# Autodesk Inventor assembly: Calorímetro
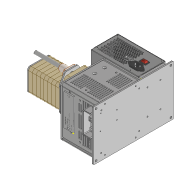
[picture p0: Inventor's stored thumbnail of the model, 180x180]
Saved by Autodesk Inventor 2020 (Build 240168000, 168)
## iProperties
Created: 2022-07-16
Part Number: Calorímetro
Document SubType Name: Assembly
Designer: gabri
Author: gabri
## Documents named in this file (15)
- C:\Users\gabri\OneDrive\Área de Trabalho\Calorimetro 2022\Calorimetro github\Inventor\Calorímetro.iam
- C:\Users\gabri\OneDrive\Área de Trabalho\Calorimetro 2022\Calorimetro github\Inventor\Fonte\ATX Power Supply v1.iam
- C:\Users\gabri\OneDrive\Área de Trabalho\Calorimetro 2022\Calorimetro github\Inventor\Base.ipt
- C:\Users\gabri\OneDrive\Área de Trabalho\Calorimetro 2022\Calorimetro github\Inventor\parte_superior.iam
- C:\Users\gabri\OneDrive\Área de Trabalho\Calorimetro 2022\Calorimetro github\Inventor\Montagem_suporte_termopar.iam
- C:\Users\gabri\OneDrive\Área de Trabalho\Calorimetro 2022\Calorimetro github\Inventor\Peça4.ipt
- C:\Users\gabri\OneDrive\Área de Trabalho\Calorimetro 2022\Calorimetro github\Inventor\suporte-fonte.ipt
- C:\Users\gabri\OneDrive\Área de Trabalho\Calorimetro 2022\Calorimetro github\Inventor\suporte_fechamento.ipt
- C:\Users\gabri\OneDrive\Área de Trabalho\Calorimetro 2022\Calorimetro github\Inventor\fechamentocima.ipt
- C:\Users\gabri\OneDrive\Área de Trabalho\Calorimetro 2022\Calorimetro github\Inventor\Mega.ipt
- C:\Users\gabri\OneDrive\Área de Trabalho\Calorimetro 2022\Calorimetro github\Inventor\suporte_fechamento_tipo2.ipt
- C:\Users\gabri\OneDrive\Área de Trabalho\Calorimetro 2022\Calorimetro github\Inventor\fechamento1.ipt
- C:\Users\gabri\OneDrive\Área de Trabalho\Calorimetro 2022\Calorimetro github\Inventor\fechamento2.ipt
- C:\Users\gabri\OneDrive\Área de Trabalho\Calorimetro 2022\Calorimetro github\Inventor\Placa.ipt
- C:\Users\gabri\OneDrive\Área de Trabalho\Calorimetro 2022\Calorimetro github\Inventor\Montagem_corpo_menor.iam
## Components (17 placed, 14 different names)
1. ATX Power Supply v1:1 [sub-assembly] — Coincidência:1, Alinhamento:1, Coincidência:2, Coincidência:5, Coincidência:6, Alinhamento:4, Alinhamento:5, Alinhamento:6, Alinhamento:7
2. Base:1 — Coincidência:7, Alinhamento:6, Alinhamento:7, Coincidência:8, Coincidência:9, Alinhamento:8, Alinhamento:9, Alinhamento:10, Coincidência:16, Alinhamento:19, Alinhamento:20, Coincidência:24
3. parte_superior:1 [sub-assembly] — Coincidência:4, Alinhamento:2, Coincidência:13, Alinhamento:17, Alinhamento:18, Coincidência:14, Coincidência:29, Coincidência:30
4. Montagem_suporte_termopar:1 [sub-assembly] — Coincidência:4, Coincidência:14, Coincidência:15, Ângulo:1
5. Peça4:1 — Alinhamento:2
6. suporte-fonte:1 — Coincidência:5, Coincidência:6, Coincidência:7, Alinhamento:4, Alinhamento:5
7. suporte_fechamento:1 — Coincidência:8, Alinhamento:8, Alinhamento:11, Alinhamento:15, Coincidência:23, Coincidência:28
8. suporte_fechamento:2 — Coincidência:9, Alinhamento:9, Alinhamento:10, Alinhamento:11, Alinhamento:16, Alinhamento:21, Alinhamento:22
9. fechamentocima:1 — Alinhamento:15, Alinhamento:16, Coincidência:13, Alinhamento:17, Alinhamento:18, Coincidência:15, Ângulo:1, Coincidência:17, Coincidência:18, Coincidência:19, Coincidência:20, Coincidência:21, Coincidência:22, Coincidência:27
10. Mega:1 — Coincidência:16, Alinhamento:19, Alinhamento:20
11. suporte_fechamento_tipo2:1 — Coincidência:17, Coincidência:18, Coincidência:19, Coincidência:26
12. suporte_fechamento:3 — Coincidência:20, Coincidência:21, Coincidência:22
13. fechamento1:1 — Alinhamento:21, Alinhamento:22
14. fechamento2:1 — Coincidência:23, Coincidência:24, Coincidência:25
15. Placa:1 — Coincidência:25
16. fechamento1:2 — Coincidência:26, Coincidência:27, Coincidência:28
17. Montagem_corpo_menor:1 [sub-assembly] — Coincidência:29, Coincidência:30
## Relationships (45: Mate 26, Flush 18, Angle 1)
- Coincidência:1 [Mate] (-71 mm): ATX Power Supply v1:1
- Alinhamento:1 [Flush]: ATX Power Supply v1:1
- Coincidência:2 [Mate]: ATX Power Supply v1:1
- Coincidência:4 [Mate]: parte_superior:1 ↔ Montagem_suporte_termopar:1
- Alinhamento:2 [Flush]: parte_superior:1 ↔ Peça4:1
- Coincidência:5 [Mate]: ATX Power Supply v1:1 ↔ suporte-fonte:1
- Coincidência:6 [Mate]: ATX Power Supply v1:1 ↔ suporte-fonte:1
- Coincidência:7 [Mate]: Base:1 ↔ suporte-fonte:1
- Alinhamento:4 [Flush]: ATX Power Supply v1:1 ↔ suporte-fonte:1
- Alinhamento:5 [Flush] (-8 mm): ATX Power Supply v1:1 ↔ suporte-fonte:1
- Alinhamento:6 [Flush] (-13 mm): ATX Power Supply v1:1 ↔ Base:1
- Alinhamento:7 [Flush]: ATX Power Supply v1:1 ↔ Base:1
- Coincidência:8 [Mate]: Base:1 ↔ suporte_fechamento:1
- Coincidência:9 [Mate]: Base:1 ↔ suporte_fechamento:2
- Alinhamento:8 [Flush]: Base:1 ↔ suporte_fechamento:1
- Alinhamento:9 [Flush]: Base:1 ↔ suporte_fechamento:2
- Alinhamento:10 [Flush] (15 mm): Base:1 ↔ suporte_fechamento:2
- Alinhamento:11 [Flush]: suporte_fechamento:1 ↔ suporte_fechamento:2
- Alinhamento:15 [Flush]: suporte_fechamento:1 ↔ fechamentocima:1
- Alinhamento:16 [Flush]: suporte_fechamento:2 ↔ fechamentocima:1
- Coincidência:13 [Mate]: parte_superior:1 ↔ fechamentocima:1
- Alinhamento:17 [Flush] (33.5 mm): parte_superior:1 ↔ fechamentocima:1
- Alinhamento:18 [Flush] (12.82 mm): parte_superior:1 ↔ fechamentocima:1
- Coincidência:14 [Mate]: parte_superior:1 ↔ Montagem_suporte_termopar:1
- Coincidência:15 [Mate]: Montagem_suporte_termopar:1 ↔ fechamentocima:1
- Ângulo:1 [Angle] (0 deg): Montagem_suporte_termopar:1 ↔ fechamentocima:1
- Coincidência:16 [Mate]: Base:1 ↔ Mega:1
- Alinhamento:19 [Flush] (3 mm): Base:1 ↔ Mega:1
- Alinhamento:20 [Flush] (26 mm): Base:1 ↔ Mega:1
- Coincidência:17 [Mate]: fechamentocima:1 ↔ suporte_fechamento_tipo2:1
- Coincidência:18 [Mate]: fechamentocima:1 ↔ suporte_fechamento_tipo2:1
- Coincidência:19 [Mate]: fechamentocima:1 ↔ suporte_fechamento_tipo2:1
- Coincidência:20 [Mate]: fechamentocima:1 ↔ suporte_fechamento:3
- Coincidência:21 [Mate]: fechamentocima:1 ↔ suporte_fechamento:3
- Coincidência:22 [Mate]: fechamentocima:1 ↔ suporte_fechamento:3
- Alinhamento:21 [Flush]: suporte_fechamento:2 ↔ fechamento1:1
- Alinhamento:22 [Flush]: suporte_fechamento:2 ↔ fechamento1:1
- Coincidência:23 [Mate]: suporte_fechamento:1 ↔ fechamento2:1
- Coincidência:24 [Mate]: Base:1 ↔ fechamento2:1
- Coincidência:25 [Mate]: fechamento2:1 ↔ Placa:1
- Coincidência:26 [Mate]: suporte_fechamento_tipo2:1 ↔ fechamento1:2
- Coincidência:27 [Mate]: fechamentocima:1 ↔ fechamento1:2
- Coincidência:28 [Mate]: suporte_fechamento:1 ↔ fechamento1:2
- Coincidência:29 [Mate]: parte_superior:1 ↔ Montagem_corpo_menor:1
- Coincidência:30 [Mate]: parte_superior:1 ↔ Montagem_corpo_menor:1
